(part 1 of 2)
# Autodesk Inventor assembly: Почти готово_CPY
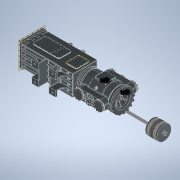
[picture p0: Inventor's stored thumbnail of the model, 180x180]
Saved by Autodesk Inventor 2021 (Build 250183000, 183)
## iProperties
Created: 2020-12-08
Part Number: Почти готово_CPY
Document SubType Name: Assembly
Designer: Тимоха
Author: Тимоха
## Documents named in this file (87)
- C:\Users\Тимоха\Desktop\КР Компрессор\compressor\Почти готово_CPY.iam
- C:\Users\Тимоха\Desktop\КР Компрессор\compressor\Фонарь_CPY.ipt
- C:\Users\Тимоха\Desktop\КР Компрессор\compressor\Башмак_CPY.ipt
- C:\Users\Тимоха\Desktop\КР Компрессор\compressor\Втулка палец шатун_CPY.ipt
- C:\Users\Тимоха\Desktop\КР Компрессор\compressor\Втулка под палец_CPY.ipt
- C:\Users\Тимоха\Desktop\КР Компрессор\compressor\Гайка шток_CPY.ipt
- C:\Users\Тимоха\Desktop\КР Компрессор\compressor\Крейцкопф_CPY.ipt
- C:\Users\Тимоха\Desktop\КР Компрессор\compressor\Палец_CPY.ipt
- C:\Users\Тимоха\Desktop\КР Компрессор\compressor\Стопорное кольцо_CPY.ipt
- C:\Users\Тимоха\Desktop\КР Компрессор\compressor\Верхняя часть поршня_CPY.ipt
- C:\Users\Тимоха\Desktop\КР Компрессор\compressor\Втулка_CPY.ipt
- C:\Users\Тимоха\Desktop\КР Компрессор\compressor\Гайка шток-поршень_CPY.ipt
- C:\Users\Тимоха\Desktop\КР Компрессор\compressor\Кольцо поршень-шток верх_CPY.ipt
- C:\Users\Тимоха\Desktop\КР Компрессор\compressor\Кольцо поршень-шток низ_CPY.ipt
- C:\Users\Тимоха\Desktop\КР Компрессор\compressor\Кольцо поршня_CPY.ipt
- C:\Users\Тимоха\Desktop\КР Компрессор\compressor\Крышка стакана_CPY.ipt
- C:\Users\Тимоха\Desktop\КР Компрессор\compressor\Крышка цилиндра 1_CPY.ipt
- C:\Users\Тимоха\Desktop\КР Компрессор\compressor\Крышка цилиндра 2_CPY.ipt
- C:\Users\Тимоха\Desktop\КР Компрессор\compressor\Нижняя часть поршня_CPY.ipt
- C:\Users\Тимоха\Desktop\КР Компрессор\compressor\Опорное кольцо_CPY.ipt
- C:\Users\Тимоха\Desktop\КР Компрессор\compressor\Цилиндр2_CPY.ipt
- C:\Users\Тимоха\Desktop\КР Компрессор\compressor\Прокладка клапана_CPY.ipt
- C:\Users\Тимоха\Desktop\КР Компрессор\compressor\Стакан1_CPY.ipt
- C:\Users\Тимоха\Desktop\КР Компрессор\compressor\Уплотнительное кольцо_CPY.ipt
- C:\Users\Тимоха\Desktop\КР Компрессор\compressor\Уплотнение фонарь_CPY.ipt
- C:\Users\Тимоха\Desktop\КР Компрессор\compressor\Корпус маслосъемника_CPY.ipt
- C:\Users\Тимоха\Desktop\КР Компрессор\compressor\Корпус сальника перегородка 1_CPY.ipt
- C:\Users\Тимоха\Desktop\КР Компрессор\compressor\Крышка перегородки11_CPY.ipt
- C:\Users\Тимоха\Desktop\КР Компрессор\compressor\Крышка перегородки12_CPY.ipt
- C:\Users\Тимоха\Desktop\КР Компрессор\compressor\Крышка перегородки21_CPY.ipt
- C:\Users\Тимоха\Desktop\КР Компрессор\compressor\Крышка перегородки22_CPY.ipt
- C:\Users\Тимоха\Desktop\КР Компрессор\compressor\Маслосъемная пружина_CPY.ipt
- C:\Users\Тимоха\Desktop\КР Компрессор\compressor\Маслосъемное кольцо_CPY.ipt
- C:\Users\Тимоха\Desktop\КР Компрессор\compressor\Придав перегородки1_CPY.ipt
- C:\Users\Тимоха\Desktop\КР Компрессор\compressor\Фланецгайка_CPY.ipt
- C:\Users\Тимоха\Desktop\КР Компрессор\compressor\Шток_CPY.ipt
- C:\Users\Тимоха\Desktop\КР Компрессор\compressor\Прокладка крейцкопф_CPY.ipt
- C:\Users\Тимоха\Documents\Inventor\Content Center Files\R2021\ru-RU\Stud GOST 22038-76\Шпилька M24-6g×70 ГОСТ 22038-76.ipt
- C:\Users\Тимоха\Documents\Inventor\Content Center Files\R2021\ru-RU\Nut GOST 15524-70\Гайка M24-6H ГОСТ 15524-70.ipt
- C:\Users\Тимоха\Documents\Inventor\Content Center Files\R2021\ru-RU\GOST 11371-78  A\Шайба 24 ГОСТ 11371-78.ipt
- C:\Users\Тимоха\Documents\Inventor\Content Center Files\R2021\ru-RU\GOST 15521-70\Гайка M20-6H ГОСТ 15521-70.ipt
- C:\Users\Тимоха\Documents\Inventor\Content Center Files\R2021\ru-RU\Stud GOST 22034-76\Шпилька M20-6g×50 ГОСТ 22034-76.ipt
- C:\Users\Тимоха\Documents\Inventor\Content Center Files\R2021\ru-RU\GOST 10450-78\Шайба 19 ГОСТ 10450-78.ipt
- C:\Users\Тимоха\Documents\Inventor\Content Center Files\R2021\ru-RU\Stud GOST 22038-76\Шпилька M20-6g×85 ГОСТ 22038-76.ipt
- C:\Users\Тимоха\Documents\Inventor\Content Center Files\R2021\ru-RU\GOST 10450-78\Шайба 21 ГОСТ 10450-78.ipt
- C:\Users\Тимоха\Documents\Inventor\Content Center Files\R2021\ru-RU\Nut GOST 15524-70\Гайка M20-6H ГОСТ 15524-70.ipt
- C:\Users\Тимоха\Documents\Inventor\Content Center Files\R2021\ru-RU\GOST 11738-84\Винт M10-6gx35 ГОСТ 11738-84.ipt
- C:\Users\Тимоха\Documents\Inventor\Content Center Files\R2021\ru-RU\GOST 11371-78  A\Шайба 12 ГОСТ 11371-78.ipt
- C:\Users\Тимоха\Documents\Inventor\Content Center Files\R2021\ru-RU\GOST 11738-84\Винт M10-6gx30 ГОСТ 11738-84.ipt
- C:\Users\Тимоха\Documents\Inventor\Content Center Files\R2021\ru-RU\GOST 11738-84\Винт M10-6gx25 ГОСТ 11738-84.ipt
- C:\Users\Тимоха\Documents\Inventor\Content Center Files\R2021\ru-RU\Stud GOST 22038-76\Шпилька M24-6g×80 ГОСТ 22038-76.ipt
- C:\Users\Тимоха\Documents\Inventor\Content Center Files\R2021\ru-RU\GOST 11371-78  A\Шайба 27 ГОСТ 11371-78.ipt
- C:\Users\Тимоха\Desktop\КР Компрессор\compressor\Крышка стакана_MIR_CPY.ipt
- C:\Users\Тимоха\Desktop\КР Компрессор\compressor\Деталь5_CPY.ipt
- C:\Users\Тимоха\Desktop\КР Компрессор\compressor\Деталь6_CPY.ipt
- C:\Users\Тимоха\Documents\Inventor\Content Center Files\R2021\ru-RU\GOST 11371-78  A\Шайба 22 ГОСТ 11371-78.ipt
- C:\Users\Тимоха\Documents\Inventor\Content Center Files\R2021\ru-RU\Bolt GOST R 50274-92\Болт M8-6g×16-F ГОСТ Р 50274-92.ipt
- C:\Users\Тимоха\Desktop\КР Компрессор\compressor\Маслоотражательное кольцо_CPY.ipt
- C:\Users\Тимоха\Desktop\КР Компрессор\compressor\Прокладка крышки фонаря 1_CPY_MIR.ipt
- C:\Users\Тимоха\Desktop\КР Компрессор\compressor\Прокладка крышки фонаря 2_CPY_MIR.ipt
- C:\Users\Тимоха\Desktop\КР Компрессор\compressor\Крышка фонаря 1.ipt
- C:\Users\Тимоха\Desktop\КР Компрессор\compressor\Крышка фонаря 2.ipt
- C:\Users\Тимоха\Desktop\КР Компрессор\compressor\Крышка фонаря 1_MIR1.ipt
- C:\Users\Тимоха\Desktop\КР Компрессор\compressor\Деталь6_CPY_MIR.ipt
- C:\Users\Тимоха\Desktop\КР Компрессор\compressor\Корпус дросселя.ipt
- C:\Users\Тимоха\Desktop\КР Компрессор\compressor\Корпус сальника 1.ipt
- C:\Users\Тимоха\Desktop\КР Компрессор\compressor\Корпус сальника 2.ipt
- C:\Users\Тимоха\Desktop\КР Компрессор\compressor\Корпус сальника 3.ipt
- C:\Users\Тимоха\Desktop\КР Компрессор\compressor\Корпус сальника 4.ipt
- C:\Users\Тимоха\Desktop\КР Компрессор\compressor\Корпус сальника0.ipt
- C:\Users\Тимоха\Desktop\КР Компрессор\compressor\Крышка сальников.ipt
- C:\Users\Тимоха\Desktop\КР Компрессор\compressor\В сальник.ipt
- C:\Users\Тимоха\Desktop\КР Компрессор\compressor\Дроссельное кольцо.ipt
- C:\Users\Тимоха\Desktop\КР Компрессор\compressor\Кольцо сальника 1.ipt
- C:\Users\Тимоха\Desktop\КР Компрессор\compressor\Кольцо сальника 2.ipt
- C:\Users\Тимоха\Desktop\КР Компрессор\compressor\Кольцо сальника.ipt
- C:\Users\Тимоха\Desktop\КР Компрессор\compressor\Пружина дросселя.ipt
- C:\Users\Тимоха\Desktop\КР Компрессор\compressor\Пружина сальника.ipt
- C:\Users\Тимоха\Desktop\КР Компрессор\compressor\Стакан2.ipt
- C:\Users\Тимоха\Desktop\КР Компрессор\compressor\Клапан 2.ipt
- C:\Users\Тимоха\Documents\Inventor\Content Center Files\R2021\ru-RU\Stud GOST 22038-76\Шпилька M12-6g×45 ГОСТ 22038-76.ipt
- C:\Users\Тимоха\Documents\Inventor\Content Center Files\R2021\ru-RU\Nut GOST 15524-70\Гайка M12-6H ГОСТ 15524-70.ipt
- C:\Users\Тимоха\Documents\Inventor\Content Center Files\R2021\ru-RU\GOST 11371-78  A\Шайба 14 ГОСТ 11371-78.ipt
- C:\Users\Тимоха\Desktop\КР Компрессор\compressor\Деталь5_CPY_MIR1.ipt
- C:\Users\Тимоха\Desktop\КР Компрессор\compressor\Клапан0.iam
- C:\Users\Тимоха\Documents\Inventor\Content Center Files\R2021\ru-RU\Stud GOST 22038-76\Шпилька M20-6g×70 ГОСТ 22038-76.ipt
- C:\Users\Тимоха\Desktop\КР Компрессор\compressor\Крышка фонаря 2_MIR2.ipt
## Components (662 placed, 86 different names)
1. Фонарь_CPY:1 — Жесткий:70, Жесткий:69, Жесткий:94, Жесткий:98, Жесткий:97, Жесткий:106, Жесткий:127, Жесткий:165, Жесткий:166, Жесткий:164, Жесткий:171, Жесткий:173, Жесткий:174, Жесткий:172, Жесткий:169, Жесткий:167, Жесткий:170, Жесткий:168, Жесткий:192, Жесткий:197, Жесткий:191, Жесткий:196, Жесткий:194, Жесткий:193, Жесткий:195, Заподлицо:9, Заподлицо:10, Заподлицо:11, Заподлицо:12, Жесткий:478, С поворотом:9, Жесткий:568, Жесткий:570, Жесткий:571
2. Башмак_CPY:1 — Жесткий:4, С поворотом:9
3. Втулка палец шатун_CPY:1 — Жесткий:3
4. Втулка под палец_CPY:1 — Жесткий:1, С поворотом:1
5. Гайка шток_CPY:1
6. Крейцкопф_CPY:1 — Жесткий:4, Жесткий:1, Жесткий:2, Жесткий:5, Жесткий:479, Жесткий:481, Жесткий:484
7. Втулка под палец_CPY:2 — Жесткий:3, Жесткий:2
8. Башмак_CPY:2 — Жесткий:5
9. Палец_CPY:1 — С поворотом:1, Жесткий:7, Жесткий:6
10. Стопорное кольцо_CPY:1 — Жесткий:7
11. Стопорное кольцо_CPY:2 — Жесткий:6
12. Втулка_CPY:1 — Жесткий:16, Жесткий:15
13. Крышка стакана_CPY:1 — Жесткий:23
14. Крышка цилиндра 1_CPY:1 — Жесткий:16, Жесткий:112
15. Крышка цилиндра 2_CPY:1 — Жесткий:70, Жесткий:79, Жесткий:61, Жесткий:125, Совмещение:3, Жесткий:565
16. Цилиндр2_CPY:1 — Заподлицо:2, Жесткий:79, Жесткий:23, Жесткий:15, Жесткий:18, Жесткий:81, Жесткий:111, Жесткий:115, Жесткий:117, Жесткий:118, Жесткий:119, Жесткий:122, Жесткий:461, Жесткий:561, Жесткий:562, Жесткий:573, Жесткий:574, Жесткий:578, Жесткий:579
17. Прокладка клапана_CPY:1 — Жесткий:18
18. Стакан1_CPY:1 — Жесткий:81
19. Уплотнительное кольцо_CPY:1 — Жесткий:61
20. Уплотнение фонарь_CPY:1 — Жесткий:69
21. Корпус маслосъемника_CPY:1 — Жесткий:104, Жесткий:554, Жесткий:560
22. Корпус сальника перегородка 1_CPY:1 — Жесткий:95, Жесткий:96, Жесткий:555, Жесткий:556
23. Крышка перегородки11_CPY:1 — Жесткий:95, Жесткий:94
24. Крышка перегородки12_CPY:1 — Жесткий:96, Жесткий:128
25. Крышка перегородки21_CPY:1 — Жесткий:104, Жесткий:98, Жесткий:105
26. Крышка перегородки22_CPY:1 — Жесткий:105, Жесткий:130
27. Придав перегородки1_CPY:1 — Жесткий:97, Жесткий:134
28. Придав перегородки1_CPY:2 — Жесткий:106, Жесткий:132
29. Шпилька ГОСТ 22038-76 M24-6g×70:2 — Жесткий:114
30. Гайка ГОСТ 15524-70 M24:2 — Жесткий:114
31. Шайба  ГОСТ 11371-78 25:2 — Совмещение:2
32. Шпилька ГОСТ 22038-76 M24-6g×70:3
33. Гайка ГОСТ 15524-70 M24:3
34. Шайба  ГОСТ 11371-78 25:3
35. Шпилька ГОСТ 22038-76 M24-6g×70:4
36. Гайка ГОСТ 15524-70 M24:4
37. Шайба  ГОСТ 11371-78 25:4
38. Шпилька ГОСТ 22038-76 M24-6g×70:5
39. Гайка ГОСТ 15524-70 M24:5
40. Шайба  ГОСТ 11371-78 25:5
41. Шпилька ГОСТ 22038-76 M24-6g×70:6
42. Гайка ГОСТ 15524-70 M24:6
43. Шайба  ГОСТ 11371-78 25:6
44. Шпилька ГОСТ 22038-76 M24-6g×70:7
45. Гайка ГОСТ 15524-70 M24:7
46. Шайба  ГОСТ 11371-78 25:7
47. Шпилька ГОСТ 22038-76 M24-6g×70:8
48. Гайка ГОСТ 15524-70 M24:8
49. Шайба  ГОСТ 11371-78 25:8
50. Шпилька ГОСТ 22038-76 M24-6g×70:9
51. Гайка ГОСТ 15524-70 M24:9
52. Шайба  ГОСТ 11371-78 25:9
53. Шпилька ГОСТ 22038-76 M24-6g×70:10
54. Гайка ГОСТ 15524-70 M24:10
55. Шайба  ГОСТ 11371-78 25:10
56. Шпилька ГОСТ 22038-76 M24-6g×70:11
57. Гайка ГОСТ 15524-70 M24:11
58. Шайба  ГОСТ 11371-78 25:11
59. Шпилька ГОСТ 22038-76 M24-6g×70:12
60. Гайка ГОСТ 15524-70 M24:12
61. Шайба  ГОСТ 11371-78 25:12
62. Шпилька ГОСТ 22038-76 M24-6g×70:13
63. Гайка ГОСТ 15524-70 M24:13
64. Шайба  ГОСТ 11371-78 25:13
65. Шпилька ГОСТ 22038-76 M24-6g×70:14
66. Гайка ГОСТ 15524-70 M24:14
67. Шайба  ГОСТ 11371-78 25:14
68. Шпилька ГОСТ 22038-76 M24-6g×70:15
69. Гайка ГОСТ 15524-70 M24:15
70. Шайба  ГОСТ 11371-78 25:15
71. Шпилька ГОСТ 22038-76 M24-6g×70:16
72. Гайка ГОСТ 15524-70 M24:16
73. Шайба  ГОСТ 11371-78 25:16
74. Шпилька ГОСТ 22038-76 M24-6g×70:17
75. Гайка ГОСТ 15524-70 M24:17
76. Шайба  ГОСТ 11371-78 25:17
77. Прокладка клапана_CPY:2 — Жесткий:115
78. Стакан1_CPY:2 — Жесткий:117
79. Крышка стакана_CPY:2 — Жесткий:118
80. Шпилька ГОСТ 22038-76 M24-6g×80:1 — Жесткий:138, Жесткий:137
81. Гайка ГОСТ 15524-70 M24:18 — Жесткий:138
82. Шайба  ГОСТ 11371-78 28:1 — Жесткий:137, Жесткий:478
83. Шпилька ГОСТ 22038-76 M24-6g×80:2 — Жесткий:140, Жесткий:139
84. Гайка ГОСТ 15524-70 M24:19 — Жесткий:140
85. Шайба  ГОСТ 11371-78 28:2 — Жесткий:139
86. Шпилька ГОСТ 22038-76 M24-6g×80:3 — Жесткий:142, Жесткий:141
87. Гайка ГОСТ 15524-70 M24:20 — Жесткий:142
88. Шайба  ГОСТ 11371-78 28:3 — Жесткий:165, Жесткий:141
89. Шпилька ГОСТ 22038-76 M24-6g×80:4 — Жесткий:144, Жесткий:143
90. Гайка ГОСТ 15524-70 M24:21 — Жесткий:144
91. Шайба  ГОСТ 11371-78 28:4 — Жесткий:166, Жесткий:143
92. Шпилька ГОСТ 22038-76 M24-6g×80:5 — Жесткий:146, Жесткий:145
93. Гайка ГОСТ 15524-70 M24:22 — Жесткий:146
94. Шайба  ГОСТ 11371-78 28:5 — Жесткий:164, Жесткий:145
95. Шпилька ГОСТ 22038-76 M24-6g×80:6 — Жесткий:148, Жесткий:147
96. Гайка ГОСТ 15524-70 M24:23 — Жесткий:148
97. Шайба  ГОСТ 11371-78 28:6 — Жесткий:171, Жесткий:147
98. Шпилька ГОСТ 22038-76 M24-6g×80:7 — Жесткий:150, Жесткий:149
99. Гайка ГОСТ 15524-70 M24:24 — Жесткий:150
100. Шайба  ГОСТ 11371-78 28:7 — Жесткий:173, Жесткий:149
101. Шпилька ГОСТ 22038-76 M24-6g×80:8 — Жесткий:152, Жесткий:151
102. Гайка ГОСТ 15524-70 M24:25 — Жесткий:152
103. Шайба  ГОСТ 11371-78 28:8 — Жесткий:174, Жесткий:151
104. Шпилька ГОСТ 22038-76 M24-6g×80:9 — Жесткий:154, Жесткий:153
105. Гайка ГОСТ 15524-70 M24:26 — Жесткий:154
106. Шайба  ГОСТ 11371-78 28:9 — Жесткий:172, Жесткий:153
107. Шпилька ГОСТ 22038-76 M24-6g×80:10 — Жесткий:156, Жесткий:155
108. Гайка ГОСТ 15524-70 M24:27 — Жесткий:156
109. Шайба  ГОСТ 11371-78 28:10 — Жесткий:169, Жесткий:155
110. Шпилька ГОСТ 22038-76 M24-6g×80:11 — Жесткий:158, Жесткий:157
111. Гайка ГОСТ 15524-70 M24:28 — Жесткий:158
112. Шайба  ГОСТ 11371-78 28:11 — Жесткий:167, Жесткий:157
113. Шпилька ГОСТ 22038-76 M24-6g×80:12 — Жесткий:160, Жесткий:159
114. Гайка ГОСТ 15524-70 M24:29 — Жесткий:160
115. Шайба  ГОСТ 11371-78 28:12 — Жесткий:170, Жесткий:159
116. Шпилька ГОСТ 22038-76 M24-6g×80:13 — Жесткий:162, Жесткий:161
117. Гайка ГОСТ 15524-70 M24:30 — Жесткий:162
118. Шайба  ГОСТ 11371-78 28:13 — Жесткий:168, Жесткий:161
119. Шпилька ГОСТ 22038-76 M24-6g×80:14 — Жесткий:176, Жесткий:175
120. Гайка ГОСТ 15524-70 M24:31 — Жесткий:176
121. Шайба  ГОСТ 11371-78 28:14 — Жесткий:192, Жесткий:175
122. Шпилька ГОСТ 22038-76 M24-6g×80:15 — Жесткий:178, Жесткий:177
123. Гайка ГОСТ 15524-70 M24:32 — Жесткий:178
124. Шайба  ГОСТ 11371-78 28:15 — Жесткий:197, Жесткий:177
125. Шпилька ГОСТ 22038-76 M24-6g×80:16 — Жесткий:180, Жесткий:179
126. Гайка ГОСТ 15524-70 M24:33 — Жесткий:180
127. Шайба  ГОСТ 11371-78 28:16 — Жесткий:191, Жесткий:179
128. Шпилька ГОСТ 22038-76 M24-6g×80:17 — Жесткий:184, Жесткий:183
129. Гайка ГОСТ 15524-70 M24:34 — Жесткий:184
130. Шайба  ГОСТ 11371-78 28:17 — Жесткий:196, Жесткий:183
131. Шпилька ГОСТ 22038-76 M24-6g×80:18 — Жесткий:186, Жесткий:185
132. Гайка ГОСТ 15524-70 M24:35 — Жесткий:186
133. Шайба  ГОСТ 11371-78 28:18 — Жесткий:194, Жесткий:185
134. Шпилька ГОСТ 22038-76 M24-6g×80:19 — Жесткий:188, Жесткий:187
135. Гайка ГОСТ 15524-70 M24:36 — Жесткий:188
136. Шайба  ГОСТ 11371-78 28:19 — Жесткий:193, Жесткий:187
137. Шпилька ГОСТ 22038-76 M24-6g×80:20 — Жесткий:190, Жесткий:189
138. Гайка ГОСТ 15524-70 M24:37 — Жесткий:190
139. Шайба  ГОСТ 11371-78 28:20 — Жесткий:195, Жесткий:189
140. Крышка стакана_MIR_CPY:1 — Жесткий:582
141. Крышка стакана_MIR_CPY:2 — Жесткий:580
142. Деталь6_CPY:2
143. Шпилька ГОСТ 22038-76 M20-6g×85:2 — Жесткий:484, Жесткий:486
144. Шпилька ГОСТ 22038-76 M20-6g×85:3 — Жесткий:481, Жесткий:483
145. Гайка ГОСТ 15524-70 M20:2 — Жесткий:483
146. Шайба  ГОСТ 11371-78 23:1 — Жесткий:482
147. Гайка ГОСТ 15524-70 M20:3 — Жесткий:486
148. Маслоотражательное кольцо_CPY:1
149. Прокладка крышки фонаря 1_CPY_MIR:1
150. Прокладка крышки фонаря 2_CPY_MIR:1
151. Крышка фонаря 1:1 — Заподлицо:9, Заподлицо:10, Жесткий:395, Жесткий:396, Жесткий:397, Жесткий:398, Жесткий:399, Жесткий:400, Жесткий:401, Жесткий:402, Жесткий:403, Жесткий:404, Жесткий:405, Жесткий:406
152. Крышка фонаря 2:1 — Заподлицо:11, Заподлицо:12, С поворотом:3, С поворотом:4, С поворотом:5, Жесткий:407, Жесткий:408, Жесткий:409, Жесткий:410, Жесткий:411, Жесткий:412, Жесткий:413, Жесткий:414, Жесткий:415, Жесткий:416, Жесткий:417, Жесткий:418, Жесткий:419, Жесткий:420, Жесткий:421, Жесткий:422, Жесткий:423, Жесткий:424, Жесткий:425, Жесткий:426, Жесткий:427
153. Болт ГОСТ Р 50274-92 M8-6g×16-F:65 — Жесткий:400
154. Болт ГОСТ Р 50274-92 M8-6g×16-F:66 — Жесткий:424
155. Болт ГОСТ Р 50274-92 M8-6g×16-F:69 — С поворотом:3
156. Болт ГОСТ Р 50274-92 M8-6g×16-F:70 — С поворотом:4
157. Болт ГОСТ Р 50274-92 M8-6g×16-F:71 — Жесткий:410
158. Болт ГОСТ Р 50274-92 M8-6g×16-F:72 — Жесткий:416
159. Болт ГОСТ Р 50274-92 M8-6g×16-F:74 — Жесткий:415
160. Болт ГОСТ Р 50274-92 M8-6g×16-F:76 — Жесткий:419
161. Болт ГОСТ Р 50274-92 M8-6g×16-F:77 — Жесткий:414
162. Болт ГОСТ Р 50274-92 M8-6g×16-F:78 — Жесткий:417
163. Болт ГОСТ Р 50274-92 M8-6g×16-F:79 — Жесткий:421
164. Болт ГОСТ Р 50274-92 M8-6g×16-F:80 — Жесткий:427
165. Болт ГОСТ Р 50274-92 M8-6g×16-F:82 — Жесткий:422
166. Болт ГОСТ Р 50274-92 M8-6g×16-F:83 — С поворотом:5
167. Болт ГОСТ Р 50274-92 M8-6g×16-F:87 — Жесткий:409
168. Болт ГОСТ Р 50274-92 M8-6g×16-F:88 — Жесткий:420
169. Болт ГОСТ Р 50274-92 M8-6g×16-F:89 — Жесткий:423
170. Болт ГОСТ Р 50274-92 M8-6g×16-F:92 — Жесткий:408
171. Болт ГОСТ Р 50274-92 M8-6g×16-F:95 — Жесткий:407
172. Болт ГОСТ Р 50274-92 M8-6g×16-F:96 — Жесткий:425
173. Болт ГОСТ Р 50274-92 M8-6g×16-F:101 — Жесткий:395
174. Болт ГОСТ Р 50274-92 M8-6g×16-F:102 — Жесткий:406
175. Болт ГОСТ Р 50274-92 M8-6g×16-F:104 — Жесткий:397
176. Болт ГОСТ Р 50274-92 M8-6g×16-F:105 — Жесткий:396
177. Болт ГОСТ Р 50274-92 M8-6g×16-F:106 — Жесткий:398
178. Болт ГОСТ Р 50274-92 M8-6g×16-F:107 — Жесткий:402
179. Болт ГОСТ Р 50274-92 M8-6g×16-F:108 — Жесткий:404
180. Болт ГОСТ Р 50274-92 M8-6g×16-F:110 — Жесткий:403
181. Болт ГОСТ Р 50274-92 M8-6g×16-F:114 — Жесткий:405
182. Болт ГОСТ Р 50274-92 M8-6g×16-F:115 — Жесткий:411
183. Болт ГОСТ Р 50274-92 M8-6g×16-F:118 — Жесткий:426
184. Болт ГОСТ Р 50274-92 M8-6g×16-F:119 — Жесткий:399
185. Болт ГОСТ Р 50274-92 M8-6g×16-F:123 — Жесткий:401
186. Болт ГОСТ Р 50274-92 M8-6g×16-F:124 — Жесткий:412
187. Болт ГОСТ Р 50274-92 M8-6g×16-F:128 — Жесткий:413
188. Болт ГОСТ Р 50274-92 M8-6g×16-F:132 — Жесткий:418
189. Болт ГОСТ Р 50274-92 M8-6g×16-F:133
190. Болт ГОСТ Р 50274-92 M8-6g×16-F:153
191. Болт ГОСТ Р 50274-92 M8-6g×16-F:154
192. Болт ГОСТ Р 50274-92 M8-6g×16-F:155
193. Болт ГОСТ Р 50274-92 M8-6g×16-F:156
194. Болт ГОСТ Р 50274-92 M8-6g×16-F:157
195. Болт ГОСТ Р 50274-92 M8-6g×16-F:158
196. Болт ГОСТ Р 50274-92 M8-6g×16-F:159
197. Болт ГОСТ Р 50274-92 M8-6g×16-F:160
198. Болт ГОСТ Р 50274-92 M8-6g×16-F:161
199. Болт ГОСТ Р 50274-92 M8-6g×16-F:164
200. Болт ГОСТ Р 50274-92 M8-6g×16-F:165
201. Болт ГОСТ Р 50274-92 M8-6g×16-F:169 — Жесткий:477
202. Болт ГОСТ Р 50274-92 M8-6g×16-F:170 — Жесткий:475
203. Болт ГОСТ Р 50274-92 M8-6g×16-F:171 — Жесткий:467
204. Болт ГОСТ Р 50274-92 M8-6g×16-F:172 — Жесткий:474
205. Болт ГОСТ Р 50274-92 M8-6g×16-F:173 — Жесткий:473
206. Болт ГОСТ Р 50274-92 M8-6g×16-F:174 — Жесткий:464
207. Болт ГОСТ Р 50274-92 M8-6g×16-F:175 — Жесткий:462
208. Болт ГОСТ Р 50274-92 M8-6g×16-F:178 — Жесткий:466
209. Болт ГОСТ Р 50274-92 M8-6g×16-F:179 — Жесткий:465
210. Болт ГОСТ Р 50274-92 M8-6g×16-F:180 — Жесткий:463
211. Болт ГОСТ Р 50274-92 M8-6g×16-F:187 — Жесткий:476
212. Болт ГОСТ Р 50274-92 M8-6g×16-F:188 — Жесткий:472
213. Болт ГОСТ Р 50274-92 M8-6g×16-F:189 — Жесткий:471
214. Болт ГОСТ Р 50274-92 M8-6g×16-F:190 — Жесткий:470
215. Болт ГОСТ Р 50274-92 M8-6g×16-F:191 — Жесткий:469
216. Болт ГОСТ Р 50274-92 M8-6g×16-F:192 — Жесткий:468
217. Деталь5_CPY:2 — Жесткий:461, Жесткий:569
218. Деталь6_CPY_MIR:1 — Жесткий:462, Жесткий:463, Жесткий:464, Жесткий:465, Жесткий:466, Жесткий:467, Жесткий:468, Жесткий:469, Жесткий:470, Жесткий:471, Жесткий:472, Жесткий:473, Жесткий:474, Жесткий:475, Жесткий:476, Жесткий:477, Жесткий:569
219. Шайба  ГОСТ 11371-78 23:4 — Жесткий:485
220. Фланецгайка_CPY:2 — Жесткий:480, Жесткий:482, Жесткий:485
221. Прокладка крейцкопф_CPY:2 — Жесткий:479, Жесткий:480
222. Корпус дросселя:1
223. Корпус сальника 1:1
224. Корпус сальника 2:1
225. Корпус сальника 3:1
226. Корпус сальника 4:1
227. Корпус сальника0:1
228. Крышка сальников:1 — Совмещение:3, Жесткий:566
229. В сальник:1
230. Дроссельное кольцо:1
231. Кольцо сальника 1:1
232. Кольцо сальника 2:1
233. Кольцо сальника:1
234. Пружина дросселя:1
235. Пружина сальника:1
236. Пружина сальника:2
237. Пружина сальника:3
238. Кольцо сальника:2
239. Пружина сальника:4
240. Кольцо сальника:3
241. Пружина сальника:5
242. Кольцо сальника:4
243. Пружина сальника:6
244. Кольцо сальника 1:2
245. Кольцо сальника 2:2
246. Кольцо сальника:5
247. Пружина сальника:7
248. Пружина сальника:8
249. Пружина сальника:9
250. Кольцо сальника:6
251. Пружина сальника:10
252. Кольцо сальника:7
253. Пружина сальника:11
254. Кольцо сальника:8
255. Пружина сальника:12
256. Кольцо сальника:9
257. Пружина сальника:13
258. Кольцо сальника:10
259. Пружина сальника:14
260. Кольцо сальника:11
261. Пружина сальника:15
262. Кольцо сальника:12
263. Пружина сальника:16
264. Кольцо сальника:13
265. Пружина сальника:17
266. Кольцо сальника:14
267. Пружина сальника:18
268. Маслосъемное кольцо_CPY:1 — Жесткий:557, Жесткий:559
269. Маслосъемное кольцо_CPY:2 — Жесткий:558, Жесткий:559, Жесткий:560
270. Маслосъемная пружина_CPY:1 — Жесткий:557
271. Маслосъемная пружина_CPY:2 — Жесткий:558
272. Кольцо сальника 1:3
273. Кольцо сальника 2:3
274. Кольцо сальника:15 — Жесткий:555
275. Пружина сальника:19
276. Пружина сальника:20
277. Пружина сальника:21
278. Кольцо сальника 1:4
279. Кольцо сальника 2:4
280. Кольцо сальника:16 — Жесткий:554
281. Пружина сальника:22
282. Пружина сальника:23
283. Пружина сальника:24
284. Кольцо сальника 1:6
285. Кольцо сальника 2:6
286. Кольцо сальника:18 — Жесткий:556
287. Пружина сальника:28
288. Пружина сальника:29
289. Пружина сальника:30
290. Стакан2:1 — Жесткий:561, Жесткий:563
291. Стакан2:2 — Жесткий:562, Жесткий:564
292. Клапан 2:1 — Жесткий:563
293. Клапан 2:2 — Жесткий:564
294. Крышка фонаря 1_MIR1:2 — Жесткий:568
295. Болт ГОСТ Р 50274-92 M8-6g×16-F:193
296. Болт ГОСТ Р 50274-92 M8-6g×16-F:194
297. Болт ГОСТ Р 50274-92 M8-6g×16-F:195
298. Болт ГОСТ Р 50274-92 M8-6g×16-F:196
299. Болт ГОСТ Р 50274-92 M8-6g×16-F:197
300. Болт ГОСТ Р 50274-92 M8-6g×16-F:198
301. Болт ГОСТ Р 50274-92 M8-6g×16-F:199
302. Болт ГОСТ Р 50274-92 M8-6g×16-F:200
303. Болт ГОСТ Р 50274-92 M8-6g×16-F:201
304. Болт ГОСТ Р 50274-92 M8-6g×16-F:202
305. Болт ГОСТ Р 50274-92 M8-6g×16-F:203
306. Болт ГОСТ Р 50274-92 M8-6g×16-F:204
307. Болт ГОСТ Р 50274-92 M8-6g×16-F:205
308. Болт ГОСТ Р 50274-92 M8-6g×16-F:206
309. Болт ГОСТ Р 50274-92 M8-6g×16-F:207
310. Болт ГОСТ Р 50274-92 M8-6g×16-F:208
311. Деталь5_CPY_MIR1:1
312. Шпилька ГОСТ 22038-76 M24-6g×80:21 — Жесткий:570
313. Гайка ГОСТ 15524-70 M24:53 — Жесткий:572
314. Шайба  ГОСТ 11371-78 28:21 — Жесткий:571, Жесткий:572
315. Клапан0:1 [sub-assembly] — Жесткий:573
316. Клапан0:2 [sub-assembly] — Жесткий:574
317. Шпилька ГОСТ 22038-76 M20-6g×85:19 — Жесткий:576
318. Шпилька ГОСТ 22038-76 M20-6g×85:20 — Жесткий:575
319. Гайка ГОСТ 15524-70 M20:19 — Жесткий:575
320. Шайба  ГОСТ 11371-78 23:5
321. Гайка ГОСТ 15524-70 M20:20 — Жесткий:576
322. Шайба  ГОСТ 11371-78 23:6
323. Крышка фонаря 2_MIR2:1 — Жесткий:584, С поворотом:10, С поворотом:11, Жесткий:585, Жесткий:586, Жесткий:587, Жесткий:588, Жесткий:589, Жесткий:590, Жесткий:591, Жесткий:592, Жесткий:593, С поворотом:12, Жесткий:594, Жесткий:595, Жесткий:596, Жесткий:597, Жесткий:598, Жесткий:599, Жесткий:600, Жесткий:601, Жесткий:602, Жесткий:603, Жесткий:604
324. Болт ГОСТ Р 50274-92 M8-6g×16-F:209 — Жесткий:584
325. Болт ГОСТ Р 50274-92 M8-6g×16-F:210 — С поворотом:10
326. Болт ГОСТ Р 50274-92 M8-6g×16-F:211 — С поворотом:11
327. Болт ГОСТ Р 50274-92 M8-6g×16-F:212 — Жесткий:585
328. Болт ГОСТ Р 50274-92 M8-6g×16-F:213 — Жесткий:586
329. Болт ГОСТ Р 50274-92 M8-6g×16-F:214 — Жесткий:587
330. Болт ГОСТ Р 50274-92 M8-6g×16-F:215 — Жесткий:588
331. Болт ГОСТ Р 50274-92 M8-6g×16-F:216 — Жесткий:589
332. Болт ГОСТ Р 50274-92 M8-6g×16-F:217 — Жесткий:590
333. Болт ГОСТ Р 50274-92 M8-6g×16-F:218 — Жесткий:591
334. Болт ГОСТ Р 50274-92 M8-6g×16-F:219 — Жесткий:592
335. Болт ГОСТ Р 50274-92 M8-6g×16-F:220 — Жесткий:593
336. Болт ГОСТ Р 50274-92 M8-6g×16-F:221 — С поворотом:12
337. Болт ГОСТ Р 50274-92 M8-6g×16-F:222 — Жесткий:594
338. Болт ГОСТ Р 50274-92 M8-6g×16-F:223 — Жесткий:595
339. Болт ГОСТ Р 50274-92 M8-6g×16-F:224 — Жесткий:596
340. Болт ГОСТ Р 50274-92 M8-6g×16-F:225 — Жесткий:597
341. Болт ГОСТ Р 50274-92 M8-6g×16-F:226 — Жесткий:598
342. Болт ГОСТ Р 50274-92 M8-6g×16-F:227 — Жесткий:599
343. Болт ГОСТ Р 50274-92 M8-6g×16-F:228 — Жесткий:600
344. Болт ГОСТ Р 50274-92 M8-6g×16-F:229 — Жесткий:601
345. Болт ГОСТ Р 50274-92 M8-6g×16-F:230 — Жесткий:602
346. Болт ГОСТ Р 50274-92 M8-6g×16-F:231 — Жесткий:603
347. Болт ГОСТ Р 50274-92 M8-6g×16-F:232 — Жесткий:604
348. Верхняя часть поршня_CPY:2
349. Гайка шток-поршень_CPY:2
350. Кольцо поршень-шток верх_CPY:2
351. Кольцо поршень-шток низ_CPY:2
352. Кольцо поршня_CPY:4
353. Нижняя часть поршня_CPY:2
354. Опорное кольцо_CPY:3
355. Кольцо поршня_CPY:5
356. Кольцо поршня_CPY:6
357. Опорное кольцо_CPY:4
358. Шток_CPY:2
359. Шпилька ГОСТ 22038-76 M20-6g×70:1 — Жесткий:126, Жесткий:125
360. Шайба ГОСТ 10450-78 21:1 — Жесткий:126
361. Гайка ГОСТ 15524-70 M20:1 — Жесткий:127
362. Шпилька ГОСТ 22038-76 M20-6g×70:2
363. Шайба ГОСТ 10450-78 21:2
364. Гайка ГОСТ 15524-70 M20:4
365. Шпилька ГОСТ 22038-76 M20-6g×70:3
366. Шайба ГОСТ 10450-78 21:3
367. Гайка ГОСТ 15524-70 M20:5
368. Шпилька ГОСТ 22038-76 M20-6g×70:4
369. Шайба ГОСТ 10450-78 21:4
370. Гайка ГОСТ 15524-70 M20:6
371. Шпилька ГОСТ 22038-76 M20-6g×70:5
372. Шайба ГОСТ 10450-78 21:5
373. Гайка ГОСТ 15524-70 M20:7
374. Шпилька ГОСТ 22038-76 M20-6g×70:6
375. Шайба ГОСТ 10450-78 21:6
376. Гайка ГОСТ 15524-70 M20:8
377. Шпилька ГОСТ 22038-76 M20-6g×70:7
378. Шайба ГОСТ 10450-78 21:7
379. Гайка ГОСТ 15524-70 M20:9
380. Шпилька ГОСТ 22038-76 M20-6g×70:8
381. Шайба ГОСТ 10450-78 21:8
382. Гайка ГОСТ 15524-70 M20:10
383. Шпилька ГОСТ 22038-76 M20-6g×70:9
384. Шайба ГОСТ 10450-78 21:9
385. Гайка ГОСТ 15524-70 M20:11
386. Шпилька ГОСТ 22038-76 M20-6g×70:10
387. Шайба ГОСТ 10450-78 21:10
388. Гайка ГОСТ 15524-70 M20:12
389. Шпилька ГОСТ 22038-76 M20-6g×70:11
390. Шайба ГОСТ 10450-78 21:11
391. Гайка ГОСТ 15524-70 M20:13
392. Шпилька ГОСТ 22038-76 M20-6g×70:12
393. Шайба ГОСТ 10450-78 21:12
394. Гайка ГОСТ 15524-70 M20:14
395. Шпилька ГОСТ 22038-76 M20-6g×70:13
396. Шайба ГОСТ 10450-78 21:13
397. Гайка ГОСТ 15524-70 M20:15
398. Шпилька ГОСТ 22038-76 M20-6g×70:14
399. Шайба ГОСТ 10450-78 21:14
400. Гайка ГОСТ 15524-70 M20:16
401. Шпилька ГОСТ 22038-76 M20-6g×70:15
402. Шайба ГОСТ 10450-78 21:15
403. Гайка ГОСТ 15524-70 M20:17
404. Шпилька ГОСТ 22038-76 M20-6g×70:16
405. Шайба ГОСТ 10450-78 21:16
406. Гайка ГОСТ 15524-70 M20:18
407. Гайка ГОСТ 15521-70 M20:1 — Жесткий:121
408. Шпилька ГОСТ 22034-76 M20-6g×50:1 — Жесткий:119, Жесткий:121, Жесткий:120
409. Шайба ГОСТ 10450-78 19:1 — Жесткий:120
410. Гайка ГОСТ 15521-70 M20:5
411. Шпилька ГОСТ 22034-76 M20-6g×50:5
412. Шайба ГОСТ 10450-78 19:5
413. Гайка ГОСТ 15521-70 M20:6
414. Шпилька ГОСТ 22034-76 M20-6g×50:6
415. Шайба ГОСТ 10450-78 19:6
416. Гайка ГОСТ 15521-70 M20:7
417. Шпилька ГОСТ 22034-76 M20-6g×50:7
418. Шайба ГОСТ 10450-78 19:7
419. Гайка ГОСТ 15521-70 M20:8
420. Шпилька ГОСТ 22034-76 M20-6g×50:8
421. Шайба ГОСТ 10450-78 19:8
422. Гайка ГОСТ 15521-70 M20:9
423. Шпилька ГОСТ 22034-76 M20-6g×50:9
424. Шайба ГОСТ 10450-78 19:9
425. Гайка ГОСТ 15521-70 M20:10
426. Шпилька ГОСТ 22034-76 M20-6g×50:10
427. Шайба ГОСТ 10450-78 19:10
428. Гайка ГОСТ 15521-70 M20:11
429. Шпилька ГОСТ 22034-76 M20-6g×50:11
430. Шайба ГОСТ 10450-78 19:11
431. Гайка ГОСТ 15521-70 M20:12
432. Шпилька ГОСТ 22034-76 M20-6g×50:12
433. Шайба ГОСТ 10450-78 19:12
434. Гайка ГОСТ 15521-70 M20:13
435. Шпилька ГОСТ 22034-76 M20-6g×50:13
436. Шайба ГОСТ 10450-78 19:13
437. Шпилька ГОСТ 22038-76 M24-6g×70:1 — Жесткий:113, Жесткий:111
438. Гайка ГОСТ 15524-70 M24:1 — Жесткий:113
439. Шайба  ГОСТ 11371-78 25:1 — Заподлицо:1, Жесткий:112
440. Шпилька ГОСТ 22038-76 M24-6g×70:18
441. Гайка ГОСТ 15524-70 M24:38
442. Шайба  ГОСТ 11371-78 25:18
443. Шпилька ГОСТ 22038-76 M24-6g×70:19
444. Гайка ГОСТ 15524-70 M24:39
445. Шайба  ГОСТ 11371-78 25:19
446. Шпилька ГОСТ 22038-76 M24-6g×70:20
447. Гайка ГОСТ 15524-70 M24:40
448. Шайба  ГОСТ 11371-78 25:20
449. Шпилька ГОСТ 22038-76 M24-6g×70:21
450. Гайка ГОСТ 15524-70 M24:41
451. Шайба  ГОСТ 11371-78 25:21
452. Шпилька ГОСТ 22038-76 M24-6g×70:22
453. Гайка ГОСТ 15524-70 M24:42
454. Шайба  ГОСТ 11371-78 25:22
455. Шпилька ГОСТ 22038-76 M24-6g×70:23
456. Гайка ГОСТ 15524-70 M24:43
457. Шайба  ГОСТ 11371-78 25:23
458. Шпилька ГОСТ 22038-76 M24-6g×70:24
459. Гайка ГОСТ 15524-70 M24:44
460. Шайба  ГОСТ 11371-78 25:24
461. Шпилька ГОСТ 22038-76 M24-6g×70:25
462. Гайка ГОСТ 15524-70 M24:45
463. Шайба  ГОСТ 11371-78 25:25
464. Шпилька ГОСТ 22038-76 M24-6g×70:26
465. Гайка ГОСТ 15524-70 M24:46
466. Шайба  ГОСТ 11371-78 25:26
467. Шпилька ГОСТ 22038-76 M24-6g×70:27
468. Гайка ГОСТ 15524-70 M24:47
469. Шайба  ГОСТ 11371-78 25:27
470. Шпилька ГОСТ 22038-76 M24-6g×70:28
471. Гайка ГОСТ 15524-70 M24:48
472. Шайба  ГОСТ 11371-78 25:28
473. Шпилька ГОСТ 22038-76 M24-6g×70:29
474. Гайка ГОСТ 15524-70 M24:49
475. Шайба  ГОСТ 11371-78 25:29
476. Шпилька ГОСТ 22038-76 M24-6g×70:30
477. Гайка ГОСТ 15524-70 M24:50
478. Шайба  ГОСТ 11371-78 25:30
479. Шпилька ГОСТ 22038-76 M24-6g×70:31
480. Гайка ГОСТ 15524-70 M24:51
481. Шайба  ГОСТ 11371-78 25:31
482. Шпилька ГОСТ 22038-76 M24-6g×70:32
483. Гайка ГОСТ 15524-70 M24:52
484. Шайба  ГОСТ 11371-78 25:32
485. Винт ГОСТ 11738-84 M 10x35:1 — Жесткий:129
486. Шайба  ГОСТ 11371-78 13:1 — Жесткий:128, Жесткий:129
487. Винт ГОСТ 11738-84 M 10x35:2
488. Шайба  ГОСТ 11371-78 13:5
489. Винт ГОСТ 11738-84 M 10x35:3
490. Шайба  ГОСТ 11371-78 13:6
491. Винт ГОСТ 11738-84 M 10x35:4
492. Шайба  ГОСТ 11371-78 13:7
493. Винт ГОСТ 11738-84 M 10x35:5
494. Шайба  ГОСТ 11371-78 13:8
495. Винт ГОСТ 11738-84 M 10x35:6
496. Шайба  ГОСТ 11371-78 13:9
497. Винт ГОСТ 11738-84 M 10x35:7
498. Шайба  ГОСТ 11371-78 13:10
499. Винт ГОСТ 11738-84 M 10x35:8
500. Шайба  ГОСТ 11371-78 13:11
501. Винт ГОСТ 11738-84 M 10x30:1 — Жесткий:131
502. Шайба  ГОСТ 11371-78 13:2 — Жесткий:130, Жесткий:131
503. Винт ГОСТ 11738-84 M 10x30:2
504. Шайба  ГОСТ 11371-78 13:12
505. Винт ГОСТ 11738-84 M 10x30:3
506. Шайба  ГОСТ 11371-78 13:13
507. Винт ГОСТ 11738-84 M 10x30:4
508. Шайба  ГОСТ 11371-78 13:14
509. Винт ГОСТ 11738-84 M 10x30:5
510. Шайба  ГОСТ 11371-78 13:15
511. Винт ГОСТ 11738-84 M 10x30:6
512. Шайба  ГОСТ 11371-78 13:16
513. Винт ГОСТ 11738-84 M 10x30:7
514. Шайба  ГОСТ 11371-78 13:17
515. Винт ГОСТ 11738-84 M 10x30:8
516. Шайба  ГОСТ 11371-78 13:18
517. Шайба  ГОСТ 11371-78 13:4 — Жесткий:134, Жесткий:135
518. Винт ГОСТ 11738-84 M 10x25:2 — Жесткий:135
519. Шайба  ГОСТ 11371-78 13:19
520. Винт ГОСТ 11738-84 M 10x25:3
521. Шайба  ГОСТ 11371-78 13:20
522. Винт ГОСТ 11738-84 M 10x25:4
523. Шайба  ГОСТ 11371-78 13:21
524. Винт ГОСТ 11738-84 M 10x25:5
525. Шайба  ГОСТ 11371-78 13:22
526. Винт ГОСТ 11738-84 M 10x25:6
527. Шайба  ГОСТ 11371-78 13:23
528. Винт ГОСТ 11738-84 M 10x25:7
529. Шайба  ГОСТ 11371-78 13:24
530. Винт ГОСТ 11738-84 M 10x25:8
531. Шайба  ГОСТ 11371-78 13:25
532. Винт ГОСТ 11738-84 M 10x25:9
533. Винт ГОСТ 11738-84 M 10x25:1 — Жесткий:133
534. Шайба  ГОСТ 11371-78 13:3 — Жесткий:133, Жесткий:132
535. Винт ГОСТ 11738-84 M 10x25:10
536. Шайба  ГОСТ 11371-78 13:26
537. Винт ГОСТ 11738-84 M 10x25:11
538. Шайба  ГОСТ 11371-78 13:27
539. Винт ГОСТ 11738-84 M 10x25:12
540. Шайба  ГОСТ 11371-78 13:28
541. Винт ГОСТ 11738-84 M 10x25:13
542. Шайба  ГОСТ 11371-78 13:29
543. Винт ГОСТ 11738-84 M 10x25:14
544. Шайба  ГОСТ 11371-78 13:30
545. Винт ГОСТ 11738-84 M 10x25:15
546. Шайба  ГОСТ 11371-78 13:31
547. Винт ГОСТ 11738-84 M 10x25:16
548. Шайба  ГОСТ 11371-78 13:32
549. Шпилька ГОСТ 22034-76 M20-6g×50:2 — Жесткий:122, Жесткий:124, Жесткий:123
550. Гайка ГОСТ 15521-70 M20:2 — Жесткий:124
551. Шайба ГОСТ 10450-78 19:2 — Жесткий:123
552. Шпилька ГОСТ 22034-76 M20-6g×50:14
553. Гайка ГОСТ 15521-70 M20:14
554. Шайба ГОСТ 10450-78 19:14
555. Шпилька ГОСТ 22034-76 M20-6g×50:15
556. Гайка ГОСТ 15521-70 M20:15
557. Шайба ГОСТ 10450-78 19:15
558. Шпилька ГОСТ 22034-76 M20-6g×50:16
559. Гайка ГОСТ 15521-70 M20:16
560. Шайба ГОСТ 10450-78 19:16
561. Шпилька ГОСТ 22034-76 M20-6g×50:17
562. Гайка ГОСТ 15521-70 M20:17
563. Шайба ГОСТ 10450-78 19:17
564. Шпилька ГОСТ 22034-76 M20-6g×50:18
565. Гайка ГОСТ 15521-70 M20:18
566. Шайба ГОСТ 10450-78 19:18
567. Шпилька ГОСТ 22034-76 M20-6g×50:19
568. Гайка ГОСТ 15521-70 M20:19
569. Шайба ГОСТ 10450-78 19:19
570. Шпилька ГОСТ 22034-76 M20-6g×50:20
571. Гайка ГОСТ 15521-70 M20:20
572. Шайба ГОСТ 10450-78 19:20
573. Шпилька ГОСТ 22034-76 M20-6g×50:21
574. Гайка ГОСТ 15521-70 M20:21
575. Шайба ГОСТ 10450-78 19:21
576. Шпилька ГОСТ 22034-76 M20-6g×50:22
577. Гайка ГОСТ 15521-70 M20:22
578. Шайба ГОСТ 10450-78 19:22
579. Шпилька ГОСТ 22038-76 M12-6g×45:1 — Жесткий:565
580. Гайка ГОСТ 15524-70 M12:1 — Жесткий:567
581. Шайба  ГОСТ 11371-78 15:1 — Жесткий:566, Жесткий:567
582. Шпилька ГОСТ 22038-76 M12-6g×45:2
583. Гайка ГОСТ 15524-70 M12:2
584. Шайба  ГОСТ 11371-78 15:2
585. Шпилька ГОСТ 22038-76 M12-6g×45:3
586. Гайка ГОСТ 15524-70 M12:3
587. Шайба  ГОСТ 11371-78 15:3
588. Шпилька ГОСТ 22038-76 M12-6g×45:4
589. Гайка ГОСТ 15524-70 M12:4
590. Шайба  ГОСТ 11371-78 15:4
591. Шпилька ГОСТ 22038-76 M12-6g×45:5
592. Гайка ГОСТ 15524-70 M12:5
593. Шайба  ГОСТ 11371-78 15:5
594. Шпилька ГОСТ 22038-76 M12-6g×45:6
595. Гайка ГОСТ 15524-70 M12:6
596. Шайба  ГОСТ 11371-78 15:6
597. Шпилька ГОСТ 22038-76 M12-6g×45:7
598. Гайка ГОСТ 15524-70 M12:7
599. Шайба  ГОСТ 11371-78 15:7
600. Шпилька ГОСТ 22038-76 M12-6g×45:8
601. Гайка ГОСТ 15524-70 M12:8
602. Шайба  ГОСТ 11371-78 15:8
603. Шпилька ГОСТ 22034-76 M20-6g×50:41 — Жесткий:579, Жесткий:581
604. Гайка ГОСТ 15521-70 M20:42 — Жесткий:581
605. Шайба ГОСТ 10450-78 19:41 — Жесткий:580
606. Шпилька ГОСТ 22034-76 M20-6g×50:43
607. Гайка ГОСТ 15521-70 M20:44
608. Шайба ГОСТ 10450-78 19:43
609. Шпилька ГОСТ 22034-76 M20-6g×50:44
610. Гайка ГОСТ 15521-70 M20:45
611. Шайба ГОСТ 10450-78 19:44
612. Шпилька ГОСТ 22034-76 M20-6g×50:45
613. Гайка ГОСТ 15521-70 M20:46
614. Шайба ГОСТ 10450-78 19:45
615. Шпилька ГОСТ 22034-76 M20-6g×50:46
616. Гайка ГОСТ 15521-70 M20:47
617. Шайба ГОСТ 10450-78 19:46
618. Шпилька ГОСТ 22034-76 M20-6g×50:47
619. Гайка ГОСТ 15521-70 M20:48
620. Шайба ГОСТ 10450-78 19:47
621. Шпилька ГОСТ 22034-76 M20-6g×50:48
622. Гайка ГОСТ 15521-70 M20:49
623. Шайба ГОСТ 10450-78 19:48
624. Шпилька ГОСТ 22034-76 M20-6g×50:49
625. Гайка ГОСТ 15521-70 M20:50
626. Шайба ГОСТ 10450-78 19:49
627. Шпилька ГОСТ 22034-76 M20-6g×50:50
628. Гайка ГОСТ 15521-70 M20:51
629. Шайба ГОСТ 10450-78 19:50
630. Шпилька ГОСТ 22034-76 M20-6g×50:51
631. Гайка ГОСТ 15521-70 M20:52
632. Шайба ГОСТ 10450-78 19:51
633. Шпилька ГОСТ 22034-76 M20-6g×50:42 — Жесткий:578, Жесткий:583
634. Гайка ГОСТ 15521-70 M20:43 — Жесткий:583
635. Шайба ГОСТ 10450-78 19:42 — Жесткий:582
636. Шпилька ГОСТ 22034-76 M20-6g×50:52
637. Гайка ГОСТ 15521-70 M20:53
638. Шайба ГОСТ 10450-78 19:52
639. Шпилька ГОСТ 22034-76 M20-6g×50:53
640. Гайка ГОСТ 15521-70 M20:54
641. Шайба ГОСТ 10450-78 19:53
642. Шпилька ГОСТ 22034-76 M20-6g×50:54
643. Гайка ГОСТ 15521-70 M20:55
644. Шайба ГОСТ 10450-78 19:54
645. Шпилька ГОСТ 22034-76 M20-6g×50:55
646. Гайка ГОСТ 15521-70 M20:56
647. Шайба ГОСТ 10450-78 19:55
648. Шпилька ГОСТ 22034-76 M20-6g×50:56
649. Гайка ГОСТ 15521-70 M20:57
650. Шайба ГОСТ 10450-78 19:56
651. Шпилька ГОСТ 22034-76 M20-6g×50:57
652. Гайка ГОСТ 15521-70 M20:58
653. Шайба ГОСТ 10450-78 19:57
654. Шпилька ГОСТ 22034-76 M20-6g×50:58
655. Гайка ГОСТ 15521-70 M20:59
656. Шайба ГОСТ 10450-78 19:58
657. Шпилька ГОСТ 22034-76 M20-6g×50:59
658. Гайка ГОСТ 15521-70 M20:60
659. Шайба ГОСТ 10450-78 19:59
660. Шпилька ГОСТ 22034-76 M20-6g×50:60
661. Гайка ГОСТ 15521-70 M20:61
662. Шайба ГОСТ 10450-78 19:60
## Component patterns: (16 elements, first: Шпилька ГОСТ 22038-76 M20-6g×70:1 + Шайба ГОСТ 10450-78 21:1 + Гайка ГОСТ 15524-70 M20:1), (10 elements, first: Гайка ГОСТ 15521-70 M20:1 + Шпилька ГОСТ 22034-76 M20-6g×50:1 + Шайба ГОСТ 10450-78 19:1), (16 elements, first: Шпилька ГОСТ 22038-76 M24-6g×70:1 + Гайка ГОСТ 15524-70 M24:1 + Шайба  ГОСТ 11371-78 25:1), (8 elements, first: Винт ГОСТ 11738-84 M 10x35:1 + Шайба  ГОСТ 11371-78 13:1), (8 elements, first: Винт ГОСТ 11738-84 M 10x30:1 + Шайба  ГОСТ 11371-78 13:2), (8 elements, first: Шайба  ГОСТ 11371-78 13:4 + Винт ГОСТ 11738-84 M 10x25:2), (8 elements, first: Винт ГОСТ 11738-84 M 10x25:1 + Шайба  ГОСТ 11371-78 13:3), (10 elements, first: Шпилька ГОСТ 22034-76 M20-6g×50:2 + Гайка ГОСТ 15521-70 M20:2 + Шайба ГОСТ 10450-78 19:2), (8 elements, first: Шпилька ГОСТ 22038-76 M12-6g×45:1 + Гайка ГОСТ 15524-70 M12:1 + Шайба  ГОСТ 11371-78 15:1), (10 elements, first: Шпилька ГОСТ 22034-76 M20-6g×50:41 + Гайка ГОСТ 15521-70 M20:42 + Шайба ГОСТ 10450-78 19:41), (10 elements, first: Шпилька ГОСТ 22034-76 M20-6g×50:42 + Гайка ГОСТ 15521-70 M20:43 + Шайба ГОСТ 10450-78 19:42)
## Relationships (301: WeldJoint 285, RevoluteJoint 8, Flush 6, Mate 2)
- Заподлицо:1 [Flush] (449.5 mm): Шайба  ГОСТ 11371-78 25:1
- Совмещение:2 [Mate] (449.5 mm): Шайба  ГОСТ 11371-78 25:2
- Заподлицо:2 [Flush] (-412.5 mm): Цилиндр2_CPY:1
- Жесткий:4 [WeldJoint]: Башмак_CPY:1 ↔ Крейцкопф_CPY:1
- Жесткий:1 [WeldJoint]: Втулка под палец_CPY:1 ↔ Крейцкопф_CPY:1
- Жесткий:3 [WeldJoint]: Втулка палец шатун_CPY:1 ↔ Втулка под палец_CPY:2
- Жесткий:2 [WeldJoint]: Крейцкопф_CPY:1 ↔ Втулка под палец_CPY:2
- Жесткий:5 [WeldJoint]: Крейцкопф_CPY:1 ↔ Башмак_CPY:2
- С поворотом:1 [RevoluteJoint]: Втулка под палец_CPY:1 ↔ Палец_CPY:1
- Жесткий:7 [WeldJoint]: Палец_CPY:1 ↔ Стопорное кольцо_CPY:1